# Autodesk Inventor assembly: Hotend 2.2
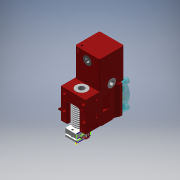
[picture p0: Inventor's stored thumbnail of the model, 180x180]
Saved by Autodesk Inventor 2018 (Build 220112000, 112)
## iProperties
Part Number: Hotend 2.2
Material: Generisch
Document SubType Name: Assembly
Designer: Till
Author: Till
## Documents named in this file (9)
- C:\Users\Till\Dropbox\Ultibox\ultibox\cad\Hotend 2.2.iam
- C:\Users\Till\Dropbox\Ultibox\ultibox\cad\Hotend Mount 2.2.ipt
- C:\Users\Till\Dropbox\Ultibox\ultibox\cad\E3D-HotEnd.iam
- C:\Users\Till\Dropbox\Ultibox\ultibox\cad\Clamp.ipt
- C:\Users\Till\Dropbox\Ultibox\ultibox\cad\LM6LUU.ipt
- C:\Users\Till\Dropbox\Ultibox\ultibox\cad\CPU - -KF0410-01.ipt
- C:\Users\Till\Dropbox\Ultibox\ultibox\cad\30mm Fan.ipt
- C:\Users\Till\Dropbox\Ultibox\ultibox\cad\fan duct 1.ipt
- C:\Users\Till\Dropbox\DIY\Stuff for other people\Sabrina\fan duct 2.ipt
## Components (9 placed, 8 different names)
1. Hotend Mount 2.2:1 — Passend:1, Passend:2, Fluchtend:1, Passend:3, Fluchtend:2, Fluchtend:3, Fluchtend:4, Fluchtend:5, Passend:6, Passend:7, Fluchtend:7, Fluchtend:8, Passend:11, Passend:12, Passend:13, Fluchtend:9, Passend:14, Passend:15, Fluchtend:10
2. E3D-HotEnd:1 [sub-assembly] — Passend:3, Fluchtend:2
3. Clamp:1 — Fluchtend:3, Fluchtend:4, Fluchtend:5, Passend:8, Passend:9, Passend:10
4. LM6LUU:1 — Passend:7, Fluchtend:7
5. LM6LUU:2 — Passend:6, Fluchtend:8
6. CPU - -KF0410-01:1 — Passend:11, Passend:12, Passend:13
7. 30mm Fan:1 — Passend:8, Passend:9, Passend:10
8. fan duct 1:1 — Fluchtend:9, Passend:14, Passend:15
9. fan duct 2:1 — Fluchtend:10
## Relationships (22: Mate 13, Flush 9)
- Passend:1 [Mate]: Hotend Mount 2.2:1
- Passend:2 [Mate]: Hotend Mount 2.2:1
- Fluchtend:1 [Flush]: Hotend Mount 2.2:1
- Passend:3 [Mate]: Hotend Mount 2.2:1 ↔ E3D-HotEnd:1
- Fluchtend:2 [Flush]: Hotend Mount 2.2:1 ↔ E3D-HotEnd:1
- Fluchtend:3 [Flush]: Hotend Mount 2.2:1 ↔ Clamp:1
- Fluchtend:4 [Flush]: Hotend Mount 2.2:1 ↔ Clamp:1
- Fluchtend:5 [Flush]: Hotend Mount 2.2:1 ↔ Clamp:1
- Passend:6 [Mate]: Hotend Mount 2.2:1 ↔ LM6LUU:2
- Passend:7 [Mate]: Hotend Mount 2.2:1 ↔ LM6LUU:1
- Fluchtend:7 [Flush]: Hotend Mount 2.2:1 ↔ LM6LUU:1
- Fluchtend:8 [Flush]: Hotend Mount 2.2:1 ↔ LM6LUU:2
- Passend:8 [Mate]: Clamp:1 ↔ 30mm Fan:1
- Passend:9 [Mate]: Clamp:1 ↔ 30mm Fan:1
- Passend:10 [Mate]: Clamp:1 ↔ 30mm Fan:1
- Passend:11 [Mate]: Hotend Mount 2.2:1 ↔ CPU - -KF0410-01:1
- Passend:12 [Mate]: Hotend Mount 2.2:1 ↔ CPU - -KF0410-01:1
- Passend:13 [Mate]: Hotend Mount 2.2:1 ↔ CPU - -KF0410-01:1
- Fluchtend:9 [Flush]: Hotend Mount 2.2:1 ↔ fan duct 1:1
- Passend:14 [Mate] (0.25 mm): Hotend Mount 2.2:1 ↔ fan duct 1:1
- Passend:15 [Mate] (0.25 mm): Hotend Mount 2.2:1 ↔ fan duct 1:1
- Fluchtend:10 [Flush]: Hotend Mount 2.2:1 ↔ fan duct 2:1
